# Autodesk Inventor assembly: VerticalElectronicsBar
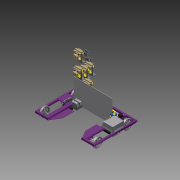
[picture p0: Inventor's stored thumbnail of the model, 180x180]
Saved by Autodesk Inventor 2012 (Build 160160000, 160)
## iProperties
Created: 2012-01-10
Part Number: VerticalElectronicsBar
Document SubType Name: Assembly
Designer: William
Author: William
## Documents named in this file (11)
- C:\Users\William\Dropbox\Robotics\CAD\team1885frc\Robot2012\Concepts\Electronics Board\VerticalElectronicsBoardDropped.iam
- C:\Users\William\Dropbox\Robotics\CAD\team1885frc\Robot2012\DriveTrain\DiveTrain_FullAssembly.iam
- C:\Users\William\Dropbox\Robotics\CAD\team1885frc\Robot2012\Concepts\Electronics Board\BatteryInMount.iam
- C:\Users\William\Dropbox\Robotics\CAD\team1885frc\Electronics\cRIO_7Slot\NI Controller.iam
- C:\Users\William\Dropbox\Robotics\CAD\team1885frc\Robot2012\Concepts\Electronics Board\DualJagSettup.iam
- C:\Users\William\Dropbox\Robotics\CAD\team1885frc\Electronics\PowerDistributionBoard\elc_Power_Distro_inv.iam
- C:\Users\William\Dropbox\Robotics\CAD\team1885frc\Electronics\DigitalSidecar\elc_Digital_Sidecar_inv.iam
- C:\Users\William\Dropbox\Robotics\CAD\team1885frc\Electronics\Breaker\Breaker.iam
- C:\Users\William\Dropbox\Robotics\CAD\team1885frc\Electronics\Spike\Spike.iam
- C:\Users\William\Dropbox\Robotics\CAD\team1885frc\Robot2012\Concepts\Electronics Board\ElectronicsBoardVerticalBottomDropped.ipt
- C:\Users\William\Dropbox\Robotics\CAD\team1885frc\Robot2012\Concepts\Electronics Board\24in-by-14inVerticalDropped.ipt
## Components (17 placed, 10 different names)
1. DiveTrain_FullAssembly:1 [sub-assembly] — Mate:1, Flush:1, Flush:2, Mate:2, Flush:3, Flush:4, Mate:6, Mate:7, Mate:8, Flush:6, Flush:7, Angle:1, Mate:10, Mate:11, Angle:2, Mate:14
2. ElectronicsBoardVerticalBottomDropped:1 — Mate:1, Flush:1, Flush:2, Mate:3, Mate:4, Flush:5, Mate:5, Mate:9, Mate:12
3. BatteryInMount:1 [sub-assembly] — Mate:2, Flush:3, Flush:4
4. DualJagSettup:1 [sub-assembly]
5. DualJagSettup:2 [sub-assembly]
6. DualJagSettup:3 [sub-assembly]
7. DualJagSettup:4 [sub-assembly]
8. DualJagSettup:5 [sub-assembly]
9. NI Controller:1 [sub-assembly] — Mate:5, Mate:6, Mate:7, Mate:13
10. Breaker:1 [sub-assembly] — Mate:8, Flush:6, Flush:7
11. elc_Digital_Sidecar_inv:1 [sub-assembly] — Mate:12, Angle:2, Mate:13, Mate:14
12. elc_Power_Distro_inv:1 [sub-assembly] — Mate:9, Angle:1, Mate:10, Mate:11
13. Spike:1 [sub-assembly]
14. Spike:2 [sub-assembly]
15. Spike:3 [sub-assembly]
16. Spike:4 [sub-assembly]
17. 24in-by-14inVerticalDropped:1 — Mate:3, Mate:4, Flush:5
## Relationships (23: Mate 14, Flush 7, Angle 2)
- Mate:1: DiveTrain_FullAssembly:1 ↔ ElectronicsBoardVerticalBottomDropped:1
- Flush:1: DiveTrain_FullAssembly:1 ↔ ElectronicsBoardVerticalBottomDropped:1
- Flush:2 (12.7 mm): DiveTrain_FullAssembly:1 ↔ ElectronicsBoardVerticalBottomDropped:1
- Mate:2: DiveTrain_FullAssembly:1 ↔ BatteryInMount:1
- Flush:3 (-12.7 mm): DiveTrain_FullAssembly:1 ↔ BatteryInMount:1
- Flush:4: DiveTrain_FullAssembly:1 ↔ BatteryInMount:1
- Mate:3: ElectronicsBoardVerticalBottomDropped:1 ↔ 24in-by-14inVerticalDropped:1
- Mate:4: ElectronicsBoardVerticalBottomDropped:1 ↔ 24in-by-14inVerticalDropped:1
- Flush:5: ElectronicsBoardVerticalBottomDropped:1 ↔ 24in-by-14inVerticalDropped:1
- Mate:5: ElectronicsBoardVerticalBottomDropped:1 ↔ NI Controller:1
- Mate:6 (12.7 mm): DiveTrain_FullAssembly:1 ↔ NI Controller:1
- Mate:7 (12.7 mm): DiveTrain_FullAssembly:1 ↔ NI Controller:1
- Mate:8: DiveTrain_FullAssembly:1 ↔ Breaker:1
- Flush:6: DiveTrain_FullAssembly:1 ↔ Breaker:1
- Flush:7 (50.8 mm): DiveTrain_FullAssembly:1 ↔ Breaker:1
- Mate:9: ElectronicsBoardVerticalBottomDropped:1 ↔ elc_Power_Distro_inv:1
- Angle:1 (180 deg): DiveTrain_FullAssembly:1 ↔ elc_Power_Distro_inv:1
- Mate:10 (50.8 mm): DiveTrain_FullAssembly:1 ↔ elc_Power_Distro_inv:1
- Mate:11 (38.1 mm): DiveTrain_FullAssembly:1 ↔ elc_Power_Distro_inv:1
- Mate:12: ElectronicsBoardVerticalBottomDropped:1 ↔ elc_Digital_Sidecar_inv:1
- Angle:2 (180 deg): DiveTrain_FullAssembly:1 ↔ elc_Digital_Sidecar_inv:1
- Mate:13 (25.4 mm): NI Controller:1 ↔ elc_Digital_Sidecar_inv:1
- Mate:14 (25.4 mm): DiveTrain_FullAssembly:1 ↔ elc_Digital_Sidecar_inv:1
